# Autodesk Inventor assembly: MDL-BDC
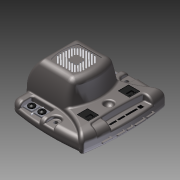
[picture p0: Inventor's stored thumbnail of the model, 180x180]
Saved by Autodesk Inventor 2015 SP1 (Build 190203100, 203)
## iProperties
Category: Control System
Company: Autodesk Inc.
Created: 2014-12-18
Part Number: MDL-BDC
Document SubType Name: Assembly
Designer: Autodesk Inc.
Catalog Web Link: http://www.ti.com/tool/mdl-bdc24?keyMatch=mdl-bdc24&tisearch=Search-EN
Vendor: Texas Instruments
Description: Motor Controller
Author: Autodesk Inc.
## Documents named in this file (4)
- D:\Data Folder\FIRST 2015\KOP_FRC\FirstChoice\CS_Controller_MDL-BDC24.iam
- D:\Data Folder\FIRST 2015\KOP_FRC\Control System\Parts\Jaguar main enclosure.ipt
- D:\Data Folder\FIRST 2015\KOP_FRC\Control System\Parts\ANSI B18.6.3 - 8-36 UNF - 0.25(7).ipt
- D:\Data Folder\FIRST 2015\KOP_FRC\Control System\Parts\IFI - 4(16).ipt
## Components (9 placed, 3 different names)
1. Jaguar main enclosure:1 — Mate:2, Mate:3
2. Cross Recessed Pan Head Machine Screw - Type II - Inch No. 8 - 36 - 1/4:1 — Mate:2, Insert:1
3. Square Test Washer (Metric) (IFI) 4:1 — Insert:1, Mate:3, Angle:1
4. Cross Recessed Pan Head Machine Screw - Type II - Inch No. 8 - 36 - 1/4:5
5. Square Test Washer (Metric) (IFI) 4:2
6. Cross Recessed Pan Head Machine Screw - Type II - Inch No. 8 - 36 - 1/4:6 — Insert:2
7. Square Test Washer (Metric) (IFI) 4:3 — Angle:2, Insert:2
8. Cross Recessed Pan Head Machine Screw - Type II - Inch No. 8 - 36 - 1/4:7
9. Square Test Washer (Metric) (IFI) 4:4
## Component patterns: (2 elements, first: Cross Recessed Pan Head Machine Screw - Type II - Inch No. 8 - 36 - 1/4:1 + Square Test Washer (Metric) (IFI) 4:1), (2 elements, first: Cross Recessed Pan Head Machine Screw - Type II - Inch No. 8 - 36 - 1/4:6 + Square Test Washer (Metric) (IFI) 4:3)
## Relationships (6: Mate 2, Insert 2, Angle 2)
- Mate:2: Jaguar main enclosure:1 ↔ Cross Recessed Pan Head Machine Screw - Type II - Inch No. 8 - 36 - 1/4:1
- Insert:1: Cross Recessed Pan Head Machine Screw - Type II - Inch No. 8 - 36 - 1/4:1 ↔ Square Test Washer (Metric) (IFI) 4:1
- Mate:3 (1.27 mm): Jaguar main enclosure:1 ↔ Square Test Washer (Metric) (IFI) 4:1
- Angle:1 (0 deg): Square Test Washer (Metric) (IFI) 4:1
- Angle:2 (0 deg): Square Test Washer (Metric) (IFI) 4:3
- Insert:2: Cross Recessed Pan Head Machine Screw - Type II - Inch No. 8 - 36 - 1/4:6 ↔ Square Test Washer (Metric) (IFI) 4:3
